# Autodesk Inventor assembly: Medium Conveyor-Belt Link
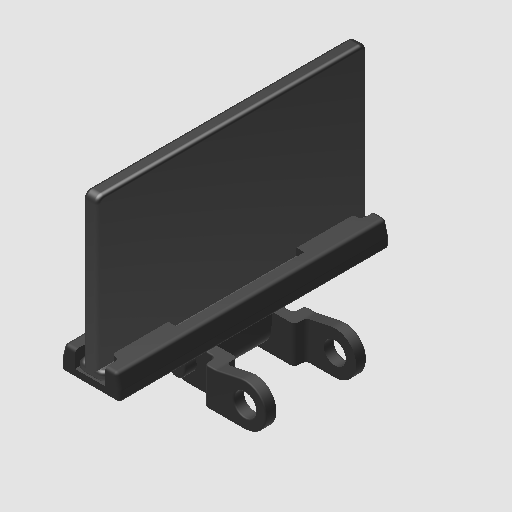
[picture p0: Inventor's stored thumbnail of the model, 512x512]
Saved by Autodesk Inventor 2019 (Build 230136000, 136)
## iProperties
Category: Motion
Company: Super Sonic Sparks, Team 24
Vendor: VEX Robotics, Inc.
Document SubType Name: Assembly
Designer: Jordan Kiesel
Catalog Web Link: vexrobotics.com/276-2214.html
Description: For use in constructing conveyor belt type mechanisms.
Created: 2018-08-26
Author: Jordan Kiesel
Title: Medium Conveyor-Belt Link
Comments: For use in constructing conveyor belt type mechanisms. ▷ Compatible with Tank Tread Kit, High Strength Chain & Sprockets.
## Documents named in this file (3)
- D:\建模\矮子机\2016 BNS CAD Library (beta)\运动\履带链条\Medium Conveyor-Belt Link.iam
- D:\建模\矮子机\2016 BNS CAD Library (beta)\运动\履带链条\Reference Parts\Conveyor-Belt Links\Conveyor-Belt Base Link.ipt
- D:\建模\矮子机\2016 BNS CAD Library (beta)\运动\履带链条\Reference Parts\Conveyor-Belt Links\Medium Conveyor-Belt Insert.ipt
## Components (2 placed, 2 different names)
1. Conveyor-Belt Base Link:1 — Mate:1, Mate:2, Flush:1
2. Medium Conveyor-Belt Insert:1 — Mate:1, Mate:2, Flush:1
## Relationships (3: Mate 2, Flush 1)
- Mate:1: Conveyor-Belt Base Link:1 ↔ Medium Conveyor-Belt Insert:1
- Mate:2: Conveyor-Belt Base Link:1 ↔ Medium Conveyor-Belt Insert:1
- Flush:1: Conveyor-Belt Base Link:1 ↔ Medium Conveyor-Belt Insert:1
